# Autodesk Inventor assembly: Robot
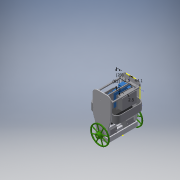
[picture p0: Inventor's stored thumbnail of the model, 180x180]
Saved by Autodesk Inventor 2019 (Build 230136000, 136)
## iProperties
Created: 2018-12-23
Part Number: Robot
Document SubType Name: Assembly
Designer: Martin
Author: Martin
## Documents named in this file (13)
- C:\Users\Martin\Projekte\Robby2\mechparts\Robot.iam
- C:\Users\Martin\Projekte\Robby2\mechparts\Motor BYGHW609.ipt
- C:\Users\Martin\Projekte\Robby2\mechparts\Wheel.ipt
- C:\Users\Martin\Projekte\Robby2\mechparts\Baseplate.ipt
- C:\Users\Martin\Projekte\Robby2\mechparts\Batteryshelf.ipt
- C:\Users\Martin\Projekte\Robby2\mechparts\Battery.ipt
- C:\Users\Martin\Projekte\Robby2\mechparts\Raspi.ipt
- C:\Users\Martin\Projekte\Robby2\mechparts\Arduino.ipt
- C:\Users\Martin\Projekte\Robby2\mechparts\Bumper.ipt
- C:\Users\Martin\Projekte\Robby2\mechparts\Sideplate right.ipt
- C:\Users\Martin\Projekte\Robby2\mechparts\Sideplate left.ipt
- C:\Users\Martin\Projekte\Robby2\mechparts\Topshelf.ipt
- C:\Users\Martin\Projekte\Robby2\mechparts\Boardcarrier.ipt
## Components (17 placed, 12 different names)
1. Sideplate right:1 — Mate:29, Mate:30, Mate:31, Mate:32, Mate:33, Mate:34, Mate:35, Mate:36, Flush:8, Mate:37, Mate:38, Mate:39, Mate:43, Mate:44, Mate:45, Mate:46, Mate:47, Mate:48, Flush:9, Mate:51, Mate:52
2. Sideplate left:1 — Mate:40, Mate:41, Mate:42, Mate:49, Mate:50, Mate:53
3. Baseplate:1 — Mate:3, Mate:4, Mate:5, Mate:6, Mate:7, Mate:8
4. Batteryshelf:1 — Mate:18, Mate:19, Mate:20, Mate:35, Mate:36, Flush:8
5. Battery:1 — Mate:18, Mate:19, Mate:20
6. Bumper:1 — Mate:37, Mate:38, Mate:39, Mate:43, Mate:44, Mate:45
7. Bumper:2 — Mate:32, Mate:33, Mate:34
8. Topshelf:1 — Mate:49, Flush:9, Mate:50
9. Boardcarrier:1 — Mate:51, Mate:52, Mate:53
10. Motor BYGHW609:1 — Mate:1, Flush:1, Mate:3, Mate:4, Mate:5, Mate:40, Mate:41, Mate:42
11. Wheel:1 — Mate:1, Flush:1
12. Motor BYGHW609:2 — Mate:2, Flush:2, Mate:6, Mate:7, Mate:8, Mate:29, Mate:30, Mate:31
13. Wheel:2 — Mate:2, Flush:2
14. Raspi:1 — Mate:21, Flush:4, Flush:5, Mate:46
15. Arduino:1 — Mate:21, Flush:4, Flush:5, Mate:47, Mate:48
16. Arduino:2 — Mate:22, Flush:6, Flush:7
17. Raspi:2 — Mate:22, Flush:6, Flush:7
## Relationships (46: Mate 38, Flush 8)
- Mate:1: Motor BYGHW609:1 ↔ Wheel:1
- Flush:1 (0.5 mm): Motor BYGHW609:1 ↔ Wheel:1
- Mate:2: Motor BYGHW609:2 ↔ Wheel:2
- Flush:2 (0.5 mm): Motor BYGHW609:2 ↔ Wheel:2
- Mate:3: Baseplate:1 ↔ Motor BYGHW609:1
- Mate:4: Baseplate:1 ↔ Motor BYGHW609:1
- Mate:5: Baseplate:1 ↔ Motor BYGHW609:1
- Mate:6: Baseplate:1 ↔ Motor BYGHW609:2
- Mate:7: Baseplate:1 ↔ Motor BYGHW609:2
- Mate:8: Baseplate:1 ↔ Motor BYGHW609:2
- Mate:18 (1 mm): Batteryshelf:1 ↔ Battery:1
- Mate:19 (0.5 mm): Batteryshelf:1 ↔ Battery:1
- Mate:20: Batteryshelf:1 ↔ Battery:1
- Mate:21 (10 mm): Raspi:1 ↔ Arduino:1
- Flush:4: Raspi:1 ↔ Arduino:1
- Flush:5: Raspi:1 ↔ Arduino:1
- Mate:22 (5 mm): Arduino:2 ↔ Raspi:2
- Flush:6: Arduino:2 ↔ Raspi:2
- Flush:7: Arduino:2 ↔ Raspi:2
- Mate:29: Sideplate right:1 ↔ Motor BYGHW609:2
- Mate:30: Sideplate right:1 ↔ Motor BYGHW609:2
- Mate:31: Sideplate right:1 ↔ Motor BYGHW609:2
- Mate:32: Sideplate right:1 ↔ Bumper:2
- Mate:33: Sideplate right:1 ↔ Bumper:2
- Mate:34: Sideplate right:1 ↔ Bumper:2
- Mate:35: Sideplate right:1 ↔ Batteryshelf:1
- Mate:36: Sideplate right:1 ↔ Batteryshelf:1
- Flush:8: Sideplate right:1 ↔ Batteryshelf:1
- Mate:37: Sideplate right:1 ↔ Bumper:1
- Mate:38: Sideplate right:1 ↔ Bumper:1
- Mate:39: Sideplate right:1 ↔ Bumper:1
- Mate:40: Sideplate left:1 ↔ Motor BYGHW609:1
- Mate:41: Sideplate left:1 ↔ Motor BYGHW609:1
- Mate:42: Sideplate left:1 ↔ Motor BYGHW609:1
- Mate:43: Sideplate right:1 ↔ Bumper:1
- Mate:44: Sideplate right:1 ↔ Bumper:1
- Mate:45: Sideplate right:1 ↔ Bumper:1
- Mate:46 (5 mm): Sideplate right:1 ↔ Raspi:1
- Mate:47: Sideplate right:1 ↔ Arduino:1
- Mate:48: Sideplate right:1 ↔ Arduino:1
- Mate:49: Sideplate left:1 ↔ Topshelf:1
- Flush:9: Sideplate right:1 ↔ Topshelf:1
- Mate:50: Sideplate left:1 ↔ Topshelf:1
- Mate:51: Sideplate right:1 ↔ Boardcarrier:1
- Mate:52: Sideplate right:1 ↔ Boardcarrier:1
- Mate:53: Sideplate left:1 ↔ Boardcarrier:1
